# Autodesk Inventor assembly: Junta tórica
Saved by Autodesk Inventor 2014 (Build 180170000, 170)
## iProperties
Created: 2014-01-28
Part Number: Junta tórica
Document SubType Name: Assembly
Designer: Sanjo
Mass: 3.39624 g
Surface Area: 43.8231 cm^2
Volume: 3.65187 cm^3
Density: 0.93 g/cm^3
ClientObjectVersion: 1
Author: Sanjo
## Documents named in this file (2)
- C:\Users\Rubén\Desktop\Robot Sumo\Piezas\Sub.Rueda\Design Accelerator\Junta tórica1.iam
- C:\Users\Sanjo\Documents\Inventor\Content Center Files\R2012\es-ES\JIS B 2406 S E\JIS 2406 - P40(3).ipt
## Components (3 placed, 1 different names)
1. JIS B 2406 estático (Externo/a) P40:1
2. JIS B 2406 estático (Externo/a) P40:2
3. JIS B 2406 estático (Externo/a) P40:3
## Component patterns: (3 elements, first: JIS B 2406 estático (Externo/a) P40:1)
